# Autodesk Inventor assembly: Arm complet v0.1
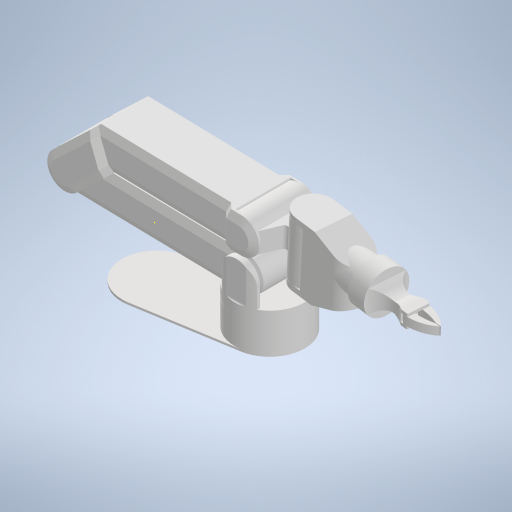
[picture p0: Inventor's stored thumbnail of the model, 512x512]
Saved by Autodesk Inventor 2023 (Build 270158000, 158)
## iProperties
Created: 2024-06-24
Part Number: Arm complet v0.1
Document SubType Name: Assembly
Designer: Swoby
Author: Swoby
## Documents named in this file (9)
- C:\Users\Swoby\OneDrive\Plocha\DUM-E\V0.1\Arm complet v0.1.iam
- C:\Users\Swoby\OneDrive\Plocha\DUM-E\V0.1\Base v0.1.ipt
- C:\Users\Swoby\OneDrive\Plocha\DUM-E\V0.1\Arm 1 v0.1.ipt
- C:\Users\Swoby\OneDrive\Plocha\DUM-E\V0.1\Arm 2 v0.1.ipt
- C:\Users\Swoby\OneDrive\Plocha\DUM-E\V0.1\Arm 3 v0.1.ipt
- C:\Users\Swoby\OneDrive\Plocha\DUM-E\V0.1\Arm 4 v0.1.ipt
- C:\Users\Swoby\OneDrive\Plocha\DUM-E\V0.1\Arm 5 v0.1.ipt
- C:\Users\Swoby\OneDrive\Plocha\DUM-E\V0.1\Arm 6 v0.1.ipt
- C:\Users\Swoby\OneDrive\Plocha\DUM-E\V0.1\Clutch.ipt
## Components (9 placed, 8 different names)
1. Base v0.1:1 — Mate:1, Mate:2
2. Arm 1 v0.1:1 — Mate:1, Mate:2, Mate:3, Mate:4
3. Arm 2 v0.1:1 — Mate:3, Mate:4, Mate:5, Mate:6
4. Arm 3 v0.1:1 — Mate:5, Mate:6, Mate:7, Mate:8
5. Arm 4 v0.1:1 — Mate:7, Mate:8, Mate:17, Mate:18
6. Arm 5 v0.1:1 — Mate:11, Mate:12, Mate:17, Mate:18
7. Arm 6 v0.1:1 — Mate:11, Mate:12, Mate:13, Mate:14, Mate:15, Mate:16
8. Clutch:1 — Mate:14, Mate:16
9. Clutch:2 — Mate:13, Mate:15
## Relationships (16: Mate 16)
- Mate:1: Base v0.1:1 ↔ Arm 1 v0.1:1
- Mate:2: Base v0.1:1 ↔ Arm 1 v0.1:1
- Mate:3: Arm 1 v0.1:1 ↔ Arm 2 v0.1:1
- Mate:4: Arm 1 v0.1:1 ↔ Arm 2 v0.1:1
- Mate:5: Arm 2 v0.1:1 ↔ Arm 3 v0.1:1
- Mate:6: Arm 2 v0.1:1 ↔ Arm 3 v0.1:1
- Mate:7: Arm 3 v0.1:1 ↔ Arm 4 v0.1:1
- Mate:8: Arm 3 v0.1:1 ↔ Arm 4 v0.1:1
- Mate:11: Arm 5 v0.1:1 ↔ Arm 6 v0.1:1
- Mate:12: Arm 5 v0.1:1 ↔ Arm 6 v0.1:1
- Mate:13: Arm 6 v0.1:1 ↔ Clutch:2
- Mate:14: Arm 6 v0.1:1 ↔ Clutch:1
- Mate:15: Arm 6 v0.1:1 ↔ Clutch:2
- Mate:16: Arm 6 v0.1:1 ↔ Clutch:1
- Mate:17: Arm 4 v0.1:1 ↔ Arm 5 v0.1:1
- Mate:18: Arm 4 v0.1:1 ↔ Arm 5 v0.1:1
